# Autodesk Inventor assembly: Apparatus Master Assem V4
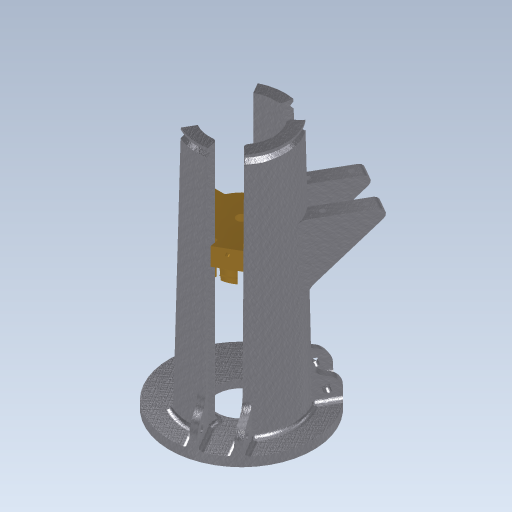
[picture p0: Inventor's stored thumbnail of the model, 512x512]
Saved by Autodesk Inventor 2023 (Build 270158000, 158)
## iProperties
Created: 2022-09-25
Part Number: Apparatus Master Assem V4
Document SubType Name: Assembly
Designer: Dave
Author: Dave
## Documents named in this file (3)
- C:\Users\Dave\Documents\GrabCAD\Chalk Bot\Chalkbot1.0\Apparatus\V4\Apparatus Master Assem V4.iam
- C:\Users\Dave\Documents\GrabCAD\Chalk Bot\Chalkbot1.0\Apparatus\V4\Slider V9 (4mm pitch).ipt
- C:\Users\Dave\Documents\GrabCAD\Chalk Bot\Chalkbot1.0\Apparatus\V4\Tower.ipt
## Components (2 placed, 2 different names)
1. Slider V8 (4mm pitch):1 — Mate:2, Angle:1
2. Tower:1 — Mate:2, Angle:1
## Relationships (2: Mate 1, Angle 1)
- Mate:2: Slider V8 (4mm pitch):1 ↔ Tower:1
- Angle:1 (0 deg): Slider V8 (4mm pitch):1 ↔ Tower:1
